# Autodesk Inventor assembly: Bar Cabinet And Base
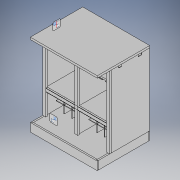
[picture p0: Inventor's stored thumbnail of the model, 180x180]
Saved by Autodesk Inventor 2016 (Build 200138000, 138)
## iProperties
Created: 2017-11-04
Part Number: Bar Cabinet And Base
Document SubType Name: Assembly
Designer: mathaetaes
Author: mathaetaes
## Documents named in this file (5)
- E:\Projects\3D Printer\printer projects\My Designs\Bar Cabinet 2.2.2018\Bar Cabinet And Base.iam
- E:\Projects\3D Printer\printer projects\My Designs\Bar Cabinet 2.2.2018\Bar Base Assembly.iam
- E:\Projects\3D Printer\printer projects\My Designs\Bar Cabinet 2.2.2018\Bar Back Cabinet.iam
- E:\Projects\3D Printer\printer projects\My Designs\Bar Cabinet 2.2.2018\Cabinet Back Sheet.ipt
- E:\Projects\3D Printer\printer projects\My Designs\Bar Cabinet 2.2.2018\Cabinet Support Frame Horizontal Bar.ipt
## Components (5 placed, 4 different names)
1. Bar Back Cabinet:1 [sub-assembly] — Mate:2, Mate:3, Mate:5, Mate:6, Mate:7, Mate:8, Mate:9, Mate:10, Mate:11, Flush:1, Mate:12, Mate:13
2. Bar Base Assembly:1 [sub-assembly] — Mate:2, Mate:3, Mate:13
3. Cabinet Back Sheet:1 — Mate:5, Mate:6, Mate:7
4. Cabinet Support Frame Horizontal Bar:1 — Mate:8, Mate:9, Mate:12
5. Cabinet Support Frame Horizontal Bar:2 — Mate:10, Mate:11, Flush:1
## Relationships (12: Mate 11, Flush 1)
- Mate:2: Bar Back Cabinet:1 ↔ Bar Base Assembly:1
- Mate:3: Bar Back Cabinet:1 ↔ Bar Base Assembly:1
- Mate:5: Bar Back Cabinet:1 ↔ Cabinet Back Sheet:1
- Mate:6: Bar Back Cabinet:1 ↔ Cabinet Back Sheet:1
- Mate:7: Bar Back Cabinet:1 ↔ Cabinet Back Sheet:1
- Mate:8: Bar Back Cabinet:1 ↔ Cabinet Support Frame Horizontal Bar:1
- Mate:9: Bar Back Cabinet:1 ↔ Cabinet Support Frame Horizontal Bar:1
- Mate:10: Bar Back Cabinet:1 ↔ Cabinet Support Frame Horizontal Bar:2
- Mate:11: Bar Back Cabinet:1 ↔ Cabinet Support Frame Horizontal Bar:2
- Flush:1 (-9.525 mm): Bar Back Cabinet:1 ↔ Cabinet Support Frame Horizontal Bar:2
- Mate:12: Bar Back Cabinet:1 ↔ Cabinet Support Frame Horizontal Bar:1
- Mate:13: Bar Back Cabinet:1 ↔ Bar Base Assembly:1
